# Autodesk Inventor assembly: enc-SidePanel Oben Links- Assembly no Absorber
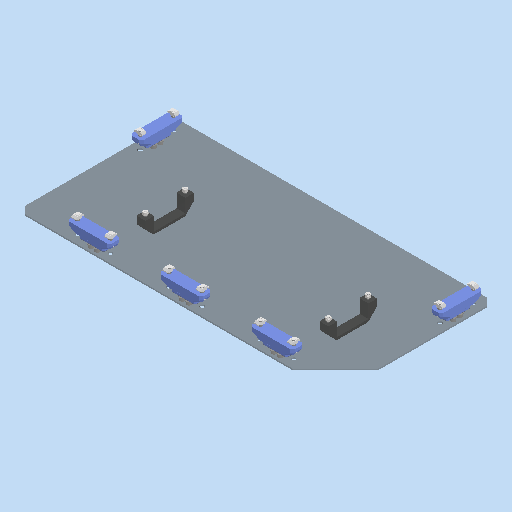
[picture p0: Inventor's stored thumbnail of the model, 512x512]
Saved by Autodesk Inventor 2023.2 (Build 272271000, 271)
## iProperties
Created: 2023-11-30
Part Number: enc-SidePanel Oben Links- Assembly no Absorber
Document SubType Name: Assembly
Designer: Nils Bade
Author: Nils Bade
## Documents named in this file (6)
- C:\Users\nilsb\Documents\Inventor\Projektarbeit-Bade\Enclosure\enc-SidePanel Oben Links - Assembly no Absorber.iam
- C:\Users\nilsb\Documents\Inventor\Projektarbeit-Bade\Enclosure\enc-SidePanel Oben 357x708.ipt
- C:\Users\nilsb\Documents\Inventor\Projektarbeit-Bade\Enclosure\V-Slot Door Handle v1.ipt
- C:\Users\nilsb\Documents\Inventor\Projektarbeit-Bade\Schrauben\Cap Head Screw M6x16 - DIN912.ipt
- C:\Users\nilsb\Documents\Inventor\Projektarbeit-Bade\RatRig_Standards\Hex Locking Nut - M6 v2.ipt
- C:\Users\nilsb\Documents\Inventor\Projektarbeit-Bade\Enclosure\Magnet PanelFrame Straight connected.iam
## Components (16 placed, 5 different names)
1. enc-SidePanel Oben 357x708:1 — Passend:1, Passend:2, Passend:3, Passend:4, Passend:5, Passend:6, Passend:7, Passend:8, Passend:19, Passend:20, Passend:21, Passend:22, Passend:23, Passend:24, Passend:25, Passend:26, Passend:27, Passend:28, Passend:29, Passend:30, Passend:31, Passend:32, Passend:33, Passend:34, Passend:35, Passend:36, Passend:37
2. V-Slot Door Handle v1:1 — Passend:1, Passend:2, Passend:3, Passend:11, Passend:12
3. V-Slot Door Handle v1:2 — Passend:4, Passend:5, Passend:6, Passend:9, Passend:10, Passend:13, Passend:14
4. Cap Head Screw M6x16 - DIN912:1 — Passend:7, Passend:12, Passend:17
5. Cap Head Screw M6x16 - DIN912:2 — Passend:8, Passend:11, Passend:18
6. Cap Head Screw M6x16 - DIN912:3 — Passend:9, Passend:13, Passend:15
7. Cap Head Screw M6x16 - DIN912:4 — Passend:10, Passend:14, Passend:16
8. Hex Locking Nut - M6 v2:1 — Passend:18, Passend:22
9. Hex Locking Nut - M6 v2:2 — Passend:17, Passend:21
10. Hex Locking Nut - M6 v2:3 — Passend:16, Passend:20
11. Hex Locking Nut - M6 v2:4 — Passend:15, Passend:19
12. Magnet PanelFrame Straight connected:1 [sub-assembly] — Passend:26, Passend:27, Passend:28
13. Magnet PanelFrame Straight connected:2 [sub-assembly] — Passend:23, Passend:24, Passend:25
14. Magnet PanelFrame Straight connected:3 [sub-assembly] — Passend:33, Passend:34, Passend:35
15. Magnet PanelFrame Straight connected:4 [sub-assembly] — Passend:31, Passend:32, Passend:36
16. Magnet PanelFrame Straight connected:5 [sub-assembly] — Passend:29, Passend:30, Passend:37
## Relationships (37: Mate 37)
- Passend:1 [Mate]: enc-SidePanel Oben 357x708:1 ↔ V-Slot Door Handle v1:1
- Passend:2 [Mate]: enc-SidePanel Oben 357x708:1 ↔ V-Slot Door Handle v1:1
- Passend:3 [Mate]: enc-SidePanel Oben 357x708:1 ↔ V-Slot Door Handle v1:1
- Passend:4 [Mate]: enc-SidePanel Oben 357x708:1 ↔ V-Slot Door Handle v1:2
- Passend:5 [Mate]: enc-SidePanel Oben 357x708:1 ↔ V-Slot Door Handle v1:2
- Passend:6 [Mate]: enc-SidePanel Oben 357x708:1 ↔ V-Slot Door Handle v1:2
- Passend:7 [Mate]: enc-SidePanel Oben 357x708:1 ↔ Cap Head Screw M6x16 - DIN912:1
- Passend:8 [Mate]: enc-SidePanel Oben 357x708:1 ↔ Cap Head Screw M6x16 - DIN912:2
- Passend:9 [Mate]: V-Slot Door Handle v1:2 ↔ Cap Head Screw M6x16 - DIN912:3
- Passend:10 [Mate]: V-Slot Door Handle v1:2 ↔ Cap Head Screw M6x16 - DIN912:4
- Passend:11 [Mate]: V-Slot Door Handle v1:1 ↔ Cap Head Screw M6x16 - DIN912:2
- Passend:12 [Mate]: V-Slot Door Handle v1:1 ↔ Cap Head Screw M6x16 - DIN912:1
- Passend:13 [Mate]: V-Slot Door Handle v1:2 ↔ Cap Head Screw M6x16 - DIN912:3
- Passend:14 [Mate]: V-Slot Door Handle v1:2 ↔ Cap Head Screw M6x16 - DIN912:4
- Passend:15 [Mate]: Cap Head Screw M6x16 - DIN912:3 ↔ Hex Locking Nut - M6 v2:4
- Passend:16 [Mate]: Cap Head Screw M6x16 - DIN912:4 ↔ Hex Locking Nut - M6 v2:3
- Passend:17 [Mate]: Cap Head Screw M6x16 - DIN912:1 ↔ Hex Locking Nut - M6 v2:2
- Passend:18 [Mate]: Cap Head Screw M6x16 - DIN912:2 ↔ Hex Locking Nut - M6 v2:1
- Passend:19 [Mate]: enc-SidePanel Oben 357x708:1 ↔ Hex Locking Nut - M6 v2:4
- Passend:20 [Mate]: enc-SidePanel Oben 357x708:1 ↔ Hex Locking Nut - M6 v2:3
- Passend:21 [Mate]: enc-SidePanel Oben 357x708:1 ↔ Hex Locking Nut - M6 v2:2
- Passend:22 [Mate]: enc-SidePanel Oben 357x708:1 ↔ Hex Locking Nut - M6 v2:1
- Passend:23 [Mate]: enc-SidePanel Oben 357x708:1 ↔ Magnet PanelFrame Straight connected:2
- Passend:24 [Mate]: enc-SidePanel Oben 357x708:1 ↔ Magnet PanelFrame Straight connected:2
- Passend:25 [Mate]: enc-SidePanel Oben 357x708:1 ↔ Magnet PanelFrame Straight connected:2
- Passend:26 [Mate]: enc-SidePanel Oben 357x708:1 ↔ Magnet PanelFrame Straight connected:1
- Passend:27 [Mate]: enc-SidePanel Oben 357x708:1 ↔ Magnet PanelFrame Straight connected:1
- Passend:28 [Mate]: enc-SidePanel Oben 357x708:1 ↔ Magnet PanelFrame Straight connected:1
- Passend:29 [Mate]: enc-SidePanel Oben 357x708:1 ↔ Magnet PanelFrame Straight connected:5
- Passend:30 [Mate]: enc-SidePanel Oben 357x708:1 ↔ Magnet PanelFrame Straight connected:5
- Passend:31 [Mate]: enc-SidePanel Oben 357x708:1 ↔ Magnet PanelFrame Straight connected:4
- Passend:32 [Mate]: enc-SidePanel Oben 357x708:1 ↔ Magnet PanelFrame Straight connected:4
- Passend:33 [Mate]: enc-SidePanel Oben 357x708:1 ↔ Magnet PanelFrame Straight connected:3
- Passend:34 [Mate]: enc-SidePanel Oben 357x708:1 ↔ Magnet PanelFrame Straight connected:3
- Passend:35 [Mate]: enc-SidePanel Oben 357x708:1 ↔ Magnet PanelFrame Straight connected:3
- Passend:36 [Mate]: enc-SidePanel Oben 357x708:1 ↔ Magnet PanelFrame Straight connected:4
- Passend:37 [Mate]: enc-SidePanel Oben 357x708:1 ↔ Magnet PanelFrame Straight connected:5
